# Autodesk Inventor assembly: 000.011 - Крепление по XT60 мама
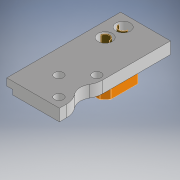
[picture p0: Inventor's stored thumbnail of the model, 180x180]
Saved by Autodesk Inventor 2022 (Build 260153000, 153)
## iProperties
Created: 2023-04-23
Part Number: 000.011 - Крепление по XT60 мама
Document SubType Name: Assembly
Designer: Иван Петров
Author: Иван Петров
## Documents named in this file (3)
- C:\Users\Ivan Petrov\Documents\GitHub\OmniBot\design\000.011 - Крепление по XT60 мама.iam
- C:\Users\Ivan Petrov\Documents\GitHub\OmniBot\design\000.011.001 - Основание.ipt
- C:\Users\Ivan Petrov\Documents\GitHub\OmniBot\design\standart_components\XT60 Buchse.ipt
## Components (2 placed, 2 different names)
1. 000.011.001 - Основание:1 — Совмещение:2, Совмещение:3, Совмещение:4
2. XT60 Buchse:1 — Совмещение:2, Совмещение:3, Совмещение:4
## Relationships (3: Mate 3)
- Совмещение:2 [Mate]: 000.011.001 - Основание:1 ↔ XT60 Buchse:1
- Совмещение:3 [Mate]: 000.011.001 - Основание:1 ↔ XT60 Buchse:1
- Совмещение:4 [Mate]: 000.011.001 - Основание:1 ↔ XT60 Buchse:1
